# Autodesk Inventor assembly: Solenoid Valve
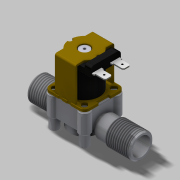
[picture p0: Inventor's stored thumbnail of the model, 180x180]
Saved by Autodesk Inventor 2020 (Build 240168000, 168)
## iProperties
Created: 2019-04-28
Part Number: Solenoid Valve
Document SubType Name: Assembly
Designer: Plo
Author: Plo
## Documents named in this file (6)
- C:\Users\LENOVO\Desktop\Graduation Project\Fish Farming Unit\Water Loop Components\Solenoid Valve.iam
- C:\Users\LENOVO\Desktop\Graduation Project\Fish Farming Unit\Water Loop Components\plastic-g1-2-solenoid-valve-1.snapshot.1\Valve.ipt
- C:\Users\LENOVO\Desktop\Graduation Project\Fish Farming Unit\Water Loop Components\plastic-g1-2-solenoid-valve-1.snapshot.1\Actuador.ipt
- C:\Users\LENOVO\Desktop\Graduation Project\Fish Farming Unit\Water Loop Components\plastic-g1-2-solenoid-valve-1.snapshot.1\Base1.ipt
- C:\Users\LENOVO\Desktop\Graduation Project\Fish Farming Unit\Water Loop Components\plastic-g1-2-solenoid-valve-1.snapshot.1\Solenoide.ipt
- C:\Users\LENOVO\Desktop\Graduation Project\Fish Farming Unit\Water Loop Components\plastic-g1-2-solenoid-valve-1.snapshot.1\Base2.ipt
## Components (5 placed, 5 different names)
1. Valve:1 — Insert:1, Angle:1
2. Actuador:1 — Insert:1, Insert:2
3. Base1:1 — Insert:2, Insert:3, Mate:1, Mate:2, Mate:3
4. Solenoide:1 — Insert:3
5. Base2:1 — Mate:1, Mate:2, Mate:3, Mate:4
## Relationships (8: Mate 4, Insert 3, Angle 1)
- Insert:1 (1 mm): Valve:1 ↔ Actuador:1
- Insert:2: Actuador:1 ↔ Base1:1
- Insert:3: Base1:1 ↔ Solenoide:1
- Mate:1: Base1:1 ↔ Base2:1
- Mate:2: Base1:1 ↔ Base2:1
- Mate:3: Base1:1 ↔ Base2:1
- Mate:4: Base2:1
- Angle:1 (0 deg): Valve:1
